# Autodesk Inventor assembly: wheel_rider
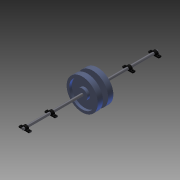
[picture p0: Inventor's stored thumbnail of the model, 180x180]
Saved by Autodesk Inventor 2011 (Build 150239000, 239)
## iProperties
Created: 2013-01-19
Part Number: wheel_rider
Document SubType Name: Assembly
Designer: Christopher
Author: Christopher
## Documents named in this file (4)
- F:\Users\Christopher\Documents\GitHub\2013CAD\2013 robot\forklift\Pneumatics and frame grabbers\wheel_rider.iam
- F:\Users\Christopher\Documents\GitHub\2013CAD\2013 robot\forklift\Misc parts\.5inch_side_bearing.ipt
- F:\Users\Christopher\Documents\GitHub\2013CAD\2013 robot\forklift\frame parts\0.5unkeyedaxle_26.ipt
- F:\Users\Christopher\Documents\GitHub\2013CAD\2013 robot\forklift\robot parts\example_wheel_6inch_.5axle.ipt
## Components (7 placed, 3 different names)
1. .5inch_side_bearing:1 — Insert:1, Flush:3
2. .5inch_side_bearing:2 — Insert:2, Flush:2, Flush:3
3. .5inch_side_bearing:3 — Insert:3, Flush:1
4. .5inch_side_bearing:4 — Insert:4, Flush:1, Flush:2
5. 0.5unkeyedaxle_26:1 — Insert:1, Insert:2, Insert:3, Insert:4, Insert:5, Insert:6
6. example_wheel_6inch_.5axle:1 — Insert:6
7. example_wheel_6inch_.5axle:2 — Insert:5
## Relationships (9: Insert 6, Flush 3)
- Insert:1 (6.35 mm): .5inch_side_bearing:1 ↔ 0.5unkeyedaxle_26:1
- Insert:2 (133.35 mm): .5inch_side_bearing:2 ↔ 0.5unkeyedaxle_26:1
- Insert:3 (6.35 mm): .5inch_side_bearing:3 ↔ 0.5unkeyedaxle_26:1
- Insert:4 (133.35 mm): .5inch_side_bearing:4 ↔ 0.5unkeyedaxle_26:1
- Flush:1: .5inch_side_bearing:3 ↔ .5inch_side_bearing:4
- Flush:2: .5inch_side_bearing:2 ↔ .5inch_side_bearing:4
- Flush:3: .5inch_side_bearing:1 ↔ .5inch_side_bearing:2
- Insert:5 (292.1 mm): 0.5unkeyedaxle_26:1 ↔ example_wheel_6inch_.5axle:2
- Insert:6 (292.1 mm): 0.5unkeyedaxle_26:1 ↔ example_wheel_6inch_.5axle:1
